# Autodesk Inventor assembly: Assembly1
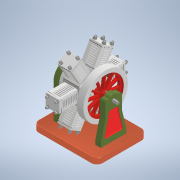
[picture p0: Inventor's stored thumbnail of the model, 180x180]
Saved by Autodesk Inventor 2020 (Build 240168000, 168)
## iProperties
Created: 2020-08-16
Part Number: Assembly1
Document SubType Name: Assembly
Designer: benny
Author: benny
## Documents named in this file (23)
- C:\Users\benny\Desktop\importantmajorprojecthev_june\engine\assembly\Assembly1.iam
- C:\Users\benny\Desktop\importantmajorprojecthev_june\engine\crankshaft assembly\crankshaft assembly.iam
- C:\Users\benny\Desktop\importantmajorprojecthev_june\engine\others\stand\stand.ipt
- C:\Users\benny\Desktop\importantmajorprojecthev_june\engine\others\bearing holder.ipt
- C:\Users\benny\Desktop\importantmajorprojecthev_june\engine\others\bearing stand without hole.ipt
- C:\Users\benny\Documents\Inventor\Content Center Files\R2020\en-US\ISO 4762(2)\ISO 4762 - M10 x 25ISO.ipt
- C:\Users\benny\Documents\Inventor\Content Center Files\R2020\en-US\Parker HB 125HBL\Parker Hose Barb to Male Pipe 125HBL 125HBL-4-2.ipt
- C:\Users\benny\Desktop\importantmajorprojecthev_june\engine\others\valve housing\valve housing.ipt
- C:\Users\benny\Desktop\importantmajorprojecthev_june\engine\others\valve\valve.ipt
- C:\Users\benny\Desktop\importantmajorprojecthev_june\engine\others\crank thing\crankcase.ipt
- C:\Users\benny\Documents\Inventor\Content Center Files\R2020\en-US\ISO 4762(2)\ISO 4762 - M6 x 45ISO.ipt
- C:\Users\benny\Desktop\importantmajorprojecthev_june\engine\assembly\Assembly2.iam
- C:\Users\benny\Documents\Inventor\Content Center Files\R2020\en-US\DIN BEARING(1)\DIN 625 SKF - SKF 6001.ipt
- C:\Users\benny\Desktop\importantmajorprojecthev_june\engine\others\connecting rod hub.ipt
- C:\Users\benny\Desktop\importantmajorprojecthev_june\engine\others\flywheel not screwed.ipt
- C:\Users\benny\Desktop\importantmajorprojecthev_june\engine\others\connecting rod.ipt
- C:\Users\benny\Desktop\importantmajorprojecthev_june\engine\piston assembly\Piston Assembly.iam
- C:\Users\benny\Documents\Inventor\Content Center Files\R2020\en-US\ISO 2338(2)\ISO 2338 - 5 h8 x 16.ipt
- C:\Users\benny\Desktop\importantmajorprojecthev_june\engine\others\crank thing\crank case cover.ipt
- C:\Users\benny\Desktop\importantmajorprojecthev_june\engine\others\crank thing\crankcase gasket.ipt
- C:\Users\benny\Documents\Inventor\Content Center Files\R2020\en-US\ISO 7045  H\ISO 7045 - M6 x 16 - 4.8 - H - ISO.ipt
- C:\Users\benny\Documents\Inventor\Content Center Files\R2020\en-US\DIN 472(2)\DIN 472 - 28x1.2.ipt
- C:\Users\benny\Documents\Inventor\Content Center Files\R2020\en-US\ISO 4028\ISO 4028 - M5 x 8 - ISO.ipt
## Components (57 placed, 22 different names)
1. crankshaft assembly:1 [sub-assembly] — Mate:93, Mate:94, Mate:95, Mate:96, Mate:97, Mate:98, Mate:117, Mate:118, Mate:119, Mate:121, Mate:128
2. stand:1 — Mate:1, Mate:2, Mate:3, Mate:4, Mate:5, Mate:6, Mate:7, Mate:8, Mate:9, Mate:10, Mate:11, Mate:12, Mate:13, Mate:14
3. bearing holder:1 — Mate:4, Mate:5, Mate:6, Mate:120, Mate:122, Mate:126
4. bearing stand without hole:1 — Mate:1, Mate:2, Mate:3, Mate:15, Mate:16, Mate:17, Mate:18, Mate:25, Mate:26, Mate:27, Mate:28, Mate:29, Mate:30, Mate:31, Mate:32, Mate:33, Mate:34, Mate:35, Mate:36
5. ISO 4762 M10 x 25:1 — Mate:11, Mate:12
6. ISO 4762 M10 x 25:2 — Mate:13, Mate:14
7. ISO 4762 M10 x 25:3 — Mate:9, Mate:10
8. ISO 4762 M10 x 25:4 — Mate:7, Mate:8
9. Parker Hose Barb to Male Pipe 125HBL 125HBL-4-2:1 — Mate:15, Mate:19
10. valve housing:1 — Mate:16, Mate:17, Mate:18, Mate:19, Mate:20, Mate:21, Mate:23, Mate:24
11. valve:1 — Mate:20, Mate:21, Mate:22, Mate:93
12. crankcase:1 — Mate:22, Mate:23, Mate:24, Mate:37, Mate:38, Mate:39, Mate:73, Mate:76, Mate:77, Mate:99, Mate:100
13. ISO 4762 M6 x 45:1 — Mate:35, Mate:36
14. ISO 4762 M6 x 45:2 — Mate:33, Mate:34
15. ISO 4762 M6 x 45:3 — Mate:31, Mate:32
16. ISO 4762 M6 x 45:4 — Mate:29, Mate:30
17. ISO 4762 M6 x 45:5 — Mate:27, Mate:28
18. ISO 4762 M6 x 45:6 — Mate:25, Mate:26
19. DIN 625 SKF SKF 6001:1 — Mate:76, Mate:77, Mate:95
20. DIN 625 SKF SKF 6001:2 — Mate:96, Mate:97
21. DIN 625 SKF SKF 6001:3 — Mate:118, Mate:119, Mate:120
22. connecting rod hub:1 — Mate:52, Mate:53, Mate:54, Mate:55, Mate:56, Mate:57, Mate:58, Mate:59, Mate:60, Mate:61, Mate:62, Mate:63, Mate:64, Mate:65, Mate:66, Mate:68, Mate:69, Flush:1, Flush:2, Flush:3, Flush:4, Flush:5, Flush:6, Mate:94
23. flywheel not screwed:1 — Mate:117, Mate:126, Mate:127
24. connecting rod:1 — Mate:56, Mate:57, Mate:83, Mate:84, Mate:85
25. connecting rod:2 — Mate:62, Mate:63, Mate:79, Mate:86
26. connecting rod:3 — Mate:60, Mate:61, Mate:78, Mate:87
27. connecting rod:4 — Mate:58, Mate:59, Mate:67, Mate:82, Mate:88
28. connecting rod:5 — Mate:52, Mate:53, Mate:89, Mate:90
29. connecting rod:6 — Mate:54, Mate:55, Mate:91, Mate:92
30. Piston Assembly:1 [sub-assembly] — Mate:82, Mate:88, Mate:124
31. Piston Assembly:2 [sub-assembly] — Mate:71, Mate:78, Mate:87
32. Piston Assembly:3 [sub-assembly] — Mate:73, Mate:83, Mate:84, Mate:85
33. Piston Assembly:4 [sub-assembly] — Mate:89, Mate:90, Mate:125
34. Piston Assembly:5 [sub-assembly] — Mate:79, Mate:86, Mate:123
35. ISO 2338 5 h8 x 16:1 — Mate:68, Flush:3
36. ISO 2338 5 h8 x 16:2 — Mate:66, Flush:5
37. ISO 2338 5 h8 x 16:3 — Mate:67, Flush:4
38. ISO 2338 5 h8 x 16:4 — Mate:65, Flush:2
39. ISO 2338 5 h8 x 16:5 — Mate:64, Flush:1
40. ISO 2338 5 h8 x 16:6 — Mate:69, Flush:6
41. Piston Assembly:6 [sub-assembly] — Mate:75, Mate:91, Mate:92
42. crank case cover:1 — Mate:98, Mate:99, Mate:100, Mate:101, Mate:102, Mate:103, Mate:104, Mate:106, Mate:107, Mate:108, Mate:109, Mate:110, Mate:111, Mate:112
43. crankcase gasket:1 — Mate:101, Mate:102, Mate:103, Mate:105, Mate:113, Mate:114, Mate:115, Mate:116
44. ISO 7045 H M6 x 16 - 4.8 - H:1 — Mate:109, Mate:112
45. ISO 7045 H M6 x 16 - 4.8 - H:2 — Mate:106, Mate:111
46. ISO 7045 H M6 x 16 - 4.8 - H:3 — Mate:110, Mate:115
47. ISO 7045 H M6 x 16 - 4.8 - H:4 — Mate:104, Mate:105, Mate:113
48. ISO 7045 H M6 x 16 - 4.8 - H:5 — Mate:107, Mate:114
49. ISO 7045 H M6 x 16 - 4.8 - H:6 — Mate:108, Mate:116
50. DIN 472 28x1.2:1 — Mate:121, Mate:122
51. ISO 4028 M5 x 8:1 — Mate:127, Mate:128
52. Assembly2:1 [sub-assembly] — Mate:37, Mate:38, Mate:39, Mate:71
53. Assembly2:7 [sub-assembly] — Mate:124
54. Assembly2:8 [sub-assembly]
55. Assembly2:9 [sub-assembly] — Mate:75
56. Assembly2:10 [sub-assembly] — Mate:125
57. Assembly2:11 [sub-assembly] — Mate:123
## Component patterns: (6 elements, first: Assembly2:1)
## Relationships (117: Mate 111, Flush 6)
- Mate:1: stand:1 ↔ bearing stand without hole:1
- Mate:2: stand:1 ↔ bearing stand without hole:1
- Mate:3: stand:1 ↔ bearing stand without hole:1
- Mate:4: stand:1 ↔ bearing holder:1
- Mate:5: stand:1 ↔ bearing holder:1
- Mate:6: stand:1 ↔ bearing holder:1
- Mate:7: stand:1 ↔ ISO 4762 M10 x 25:4
- Mate:8: stand:1 ↔ ISO 4762 M10 x 25:4
- Mate:9: stand:1 ↔ ISO 4762 M10 x 25:3
- Mate:10: stand:1 ↔ ISO 4762 M10 x 25:3
- Mate:11: stand:1 ↔ ISO 4762 M10 x 25:1
- Mate:12: stand:1 ↔ ISO 4762 M10 x 25:1
- Mate:13: stand:1 ↔ ISO 4762 M10 x 25:2
- Mate:14: stand:1 ↔ ISO 4762 M10 x 25:2
- Mate:15: bearing stand without hole:1 ↔ Parker Hose Barb to Male Pipe 125HBL 125HBL-4-2:1
- Mate:16: bearing stand without hole:1 ↔ valve housing:1
- Mate:17: bearing stand without hole:1 ↔ valve housing:1
- Mate:18: bearing stand without hole:1 ↔ valve housing:1
- Mate:19: Parker Hose Barb to Male Pipe 125HBL 125HBL-4-2:1 ↔ valve housing:1
- Mate:20: valve housing:1 ↔ valve:1
- Mate:21: valve housing:1 ↔ valve:1
- Mate:22: valve:1 ↔ crankcase:1
- Mate:23: valve housing:1 ↔ crankcase:1
- Mate:24: valve housing:1 ↔ crankcase:1
- Mate:25: bearing stand without hole:1 ↔ ISO 4762 M6 x 45:6
- Mate:26: bearing stand without hole:1 ↔ ISO 4762 M6 x 45:6
- Mate:27: bearing stand without hole:1 ↔ ISO 4762 M6 x 45:5
- Mate:28: bearing stand without hole:1 ↔ ISO 4762 M6 x 45:5
- Mate:29: bearing stand without hole:1 ↔ ISO 4762 M6 x 45:4
- Mate:30: bearing stand without hole:1 ↔ ISO 4762 M6 x 45:4
- Mate:31: bearing stand without hole:1 ↔ ISO 4762 M6 x 45:3
- Mate:32: bearing stand without hole:1 ↔ ISO 4762 M6 x 45:3
- Mate:33: bearing stand without hole:1 ↔ ISO 4762 M6 x 45:2
- Mate:34: bearing stand without hole:1 ↔ ISO 4762 M6 x 45:2
- Mate:35: bearing stand without hole:1 ↔ ISO 4762 M6 x 45:1
- Mate:36: bearing stand without hole:1 ↔ ISO 4762 M6 x 45:1
- Mate:37: crankcase:1 ↔ Assembly2:1
- Mate:38: crankcase:1 ↔ Assembly2:1
- Mate:39: crankcase:1 ↔ Assembly2:1
- Mate:52: connecting rod hub:1 ↔ connecting rod:5
- Mate:53: connecting rod hub:1 ↔ connecting rod:5
- Mate:54: connecting rod hub:1 ↔ connecting rod:6
- Mate:55: connecting rod hub:1 ↔ connecting rod:6
- Mate:56: connecting rod hub:1 ↔ connecting rod:1
- Mate:57: connecting rod hub:1 ↔ connecting rod:1
- Mate:58: connecting rod hub:1 ↔ connecting rod:4
- Mate:59: connecting rod hub:1 ↔ connecting rod:4
- Mate:60: connecting rod hub:1 ↔ connecting rod:3
- Mate:61: connecting rod hub:1 ↔ connecting rod:3
- Mate:62: connecting rod hub:1 ↔ connecting rod:2
- Mate:63: connecting rod hub:1 ↔ connecting rod:2
- Mate:64: connecting rod hub:1 ↔ ISO 2338 5 h8 x 16:5
- Mate:65: connecting rod hub:1 ↔ ISO 2338 5 h8 x 16:4
- Mate:66: connecting rod hub:1 ↔ ISO 2338 5 h8 x 16:2
- Mate:67: connecting rod:4 ↔ ISO 2338 5 h8 x 16:3
- Mate:68: connecting rod hub:1 ↔ ISO 2338 5 h8 x 16:1
- Mate:69: connecting rod hub:1 ↔ ISO 2338 5 h8 x 16:6
- Flush:1: connecting rod hub:1 ↔ ISO 2338 5 h8 x 16:5
- Flush:2: connecting rod hub:1 ↔ ISO 2338 5 h8 x 16:4
- Flush:3: connecting rod hub:1 ↔ ISO 2338 5 h8 x 16:1
- Flush:4: connecting rod hub:1 ↔ ISO 2338 5 h8 x 16:3
- Flush:5: connecting rod hub:1 ↔ ISO 2338 5 h8 x 16:2
- Flush:6: connecting rod hub:1 ↔ ISO 2338 5 h8 x 16:6
- Mate:71: Piston Assembly:2 ↔ Assembly2:1
- Mate:73: crankcase:1 ↔ Piston Assembly:3
- Mate:75: Piston Assembly:6 ↔ Assembly2:9
- Mate:76: crankcase:1 ↔ DIN 625 SKF SKF 6001:1
- Mate:77: crankcase:1 ↔ DIN 625 SKF SKF 6001:1
- Mate:78 (-5 mm): connecting rod:3 ↔ Piston Assembly:2
- Mate:79 (-5 mm): connecting rod:2 ↔ Piston Assembly:5
- Mate:82 (-5 mm): connecting rod:4 ↔ Piston Assembly:1
- Mate:83 (-5 mm): connecting rod:1 ↔ Piston Assembly:3
- Mate:84 (-5 mm): connecting rod:1 ↔ Piston Assembly:3
- Mate:85: connecting rod:1 ↔ Piston Assembly:3
- Mate:86: connecting rod:2 ↔ Piston Assembly:5
- Mate:87: connecting rod:3 ↔ Piston Assembly:2
- Mate:88: connecting rod:4 ↔ Piston Assembly:1
- Mate:89 (-5 mm): connecting rod:5 ↔ Piston Assembly:4
- Mate:90: connecting rod:5 ↔ Piston Assembly:4
- Mate:91 (-5 mm): connecting rod:6 ↔ Piston Assembly:6
- Mate:92: connecting rod:6 ↔ Piston Assembly:6
- Mate:93: crankshaft assembly:1 ↔ valve:1
- Mate:94: crankshaft assembly:1 ↔ connecting rod hub:1
- Mate:95: crankshaft assembly:1 ↔ DIN 625 SKF SKF 6001:1
- Mate:96: crankshaft assembly:1 ↔ DIN 625 SKF SKF 6001:2
- Mate:97: crankshaft assembly:1 ↔ DIN 625 SKF SKF 6001:2
- Mate:98: crankshaft assembly:1 ↔ crank case cover:1
- Mate:99: crankcase:1 ↔ crank case cover:1
- Mate:100: crankcase:1 ↔ crank case cover:1
- Mate:101: crank case cover:1 ↔ crankcase gasket:1
- Mate:102: crank case cover:1 ↔ crankcase gasket:1
- Mate:103: crank case cover:1 ↔ crankcase gasket:1
- Mate:104: crank case cover:1 ↔ ISO 7045 H M6 x 16 - 4.8 - H:4
- Mate:105: crankcase gasket:1 ↔ ISO 7045 H M6 x 16 - 4.8 - H:4
- Mate:106: crank case cover:1 ↔ ISO 7045 H M6 x 16 - 4.8 - H:2
- Mate:107: crank case cover:1 ↔ ISO 7045 H M6 x 16 - 4.8 - H:5
- Mate:108: crank case cover:1 ↔ ISO 7045 H M6 x 16 - 4.8 - H:6
- Mate:109: crank case cover:1 ↔ ISO 7045 H M6 x 16 - 4.8 - H:1
- Mate:110: crank case cover:1 ↔ ISO 7045 H M6 x 16 - 4.8 - H:3
- Mate:111: crank case cover:1 ↔ ISO 7045 H M6 x 16 - 4.8 - H:2
- Mate:112: crank case cover:1 ↔ ISO 7045 H M6 x 16 - 4.8 - H:1
- Mate:113: crankcase gasket:1 ↔ ISO 7045 H M6 x 16 - 4.8 - H:4
- Mate:114: crankcase gasket:1 ↔ ISO 7045 H M6 x 16 - 4.8 - H:5
- Mate:115: crankcase gasket:1 ↔ ISO 7045 H M6 x 16 - 4.8 - H:3
- Mate:116: crankcase gasket:1 ↔ ISO 7045 H M6 x 16 - 4.8 - H:6
- Mate:117: crankshaft assembly:1 ↔ flywheel not screwed:1
- Mate:118: crankshaft assembly:1 ↔ DIN 625 SKF SKF 6001:3
- Mate:119: crankshaft assembly:1 ↔ DIN 625 SKF SKF 6001:3
- Mate:120: bearing holder:1 ↔ DIN 625 SKF SKF 6001:3
- Mate:121: crankshaft assembly:1 ↔ DIN 472 28x1.2:1
- Mate:122: bearing holder:1 ↔ DIN 472 28x1.2:1
- Mate:123: Piston Assembly:5 ↔ Assembly2:11
- Mate:124: Piston Assembly:1 ↔ Assembly2:7
- Mate:125: Piston Assembly:4 ↔ Assembly2:10
- Mate:126 (2.5 mm): bearing holder:1 ↔ flywheel not screwed:1
- Mate:127: flywheel not screwed:1 ↔ ISO 4028 M5 x 8:1
- Mate:128 (6 mm): crankshaft assembly:1 ↔ ISO 4028 M5 x 8:1
